# Autodesk Inventor assembly: ASY MSC 100 cone
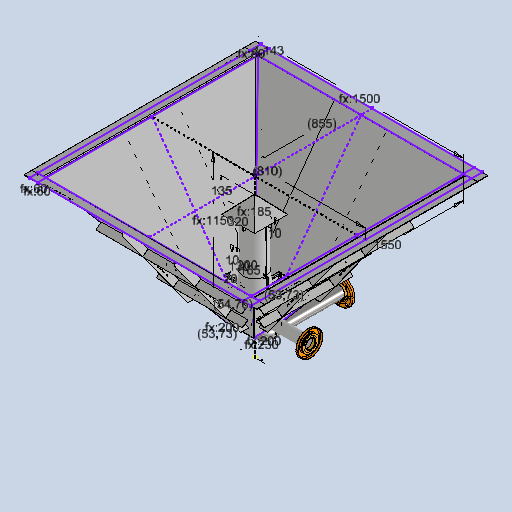
[picture p0: Inventor's stored thumbnail of the model, 512x512]
Saved by Autodesk Inventor 2025 (Build 290162010, 162A)
## iProperties
Created: 2024-05-19
Part Number: ASY MSC 100 cone
Document SubType Name: Assembly
Designer: admin
Mass: 170206 g
Surface Area: 120081 cm^2
Volume: 21304.1 cm^3
Density: 7.98935 g/cm^3
Stock Number: ASY МОО 100 конус
Author: admin
## Documents named in this file (17)
- C:\Users\pokla\Documents\Inventor\Отстойник осветлитель\Manturovo_Se-clar-Gleb\ASY MSC 100 cone.iam
- C:\Users\pokla\Documents\Inventor\Отстойник осветлитель\Manturovo_Se-clar-Gleb\MSC 114 cone IN right board.ipt
- C:\Users\pokla\Documents\Inventor\Отстойник осветлитель\Manturovo_Se-clar-Gleb\MSC 111 cone IN bottom.ipt
- C:\Users\pokla\Documents\Inventor\Отстойник осветлитель\Manturovo_Se-clar-Gleb\MSC 113 cone IN left board.ipt
- C:\Users\pokla\Documents\Inventor\Отстойник осветлитель\Manturovo_Se-clar-Gleb\MSC 112 cone IN back.ipt
- C:\Users\pokla\Documents\Inventor\Отстойник осветлитель\Manturovo_Se-clar-Gleb\MSC DIM 001 cone sketch.ipt
- C:\Users\pokla\Documents\Inventor\Отстойник осветлитель\Manturovo_Se-clar-Gleb\MSC 115 cone IN bow.ipt
- C:\Users\pokla\Documents\Inventor\Отстойник осветлитель\Manturovo_Se-clar-Gleb\MSC 110 stringer cone.ipt
- C:\Users\pokla\Documents\Inventor\Отстойник осветлитель\Manturovo_Se-clar-Gleb\MSC 106 rib cone.ipt
- C:\Users\pokla\Documents\Inventor\Отстойник осветлитель\Manturovo_Se-clar-Gleb\MSC 107 rib cone.ipt
- C:\Users\pokla\Documents\Inventor\Отстойник осветлитель\Manturovo_Se-clar-Gleb\MSC 108 rib cone.ipt
- C:\Users\pokla\Documents\Inventor\Отстойник осветлитель\Manturovo_Se-clar-Gleb\MSC 109 rib cone.ipt
- C:\Users\pokla\Documents\Inventor\Отстойник осветлитель\Manturovo_Se-clar-Gleb\ASY MSC 100.2 Cone tube.iam
- C:\Users\pokla\Documents\Inventor\Отстойник осветлитель\Manturovo_Se-clar-Gleb\ASY MSC 100.1 roсket.iam
- C:\Users\pokla\Documents\Inventor\Отстойник осветлитель\Manturovo_Se-clar-Gleb\MSC 116 rocket tube 8.ipt
- C:\Users\pokla\Documents\Inventor\Отстойник осветлитель\Manturovo_Se-clar-Gleb\Stamp flange DIN2642-065.ipt
- C:\Users\pokla\Documents\Inventor\Отстойник осветлитель\Manturovo_Se-clar-Gleb\3d party\Stamp flange DIN2642\Stamd flange lapped collar DIN2642.ipt
## Components (26 placed, 15 different names)
1. MSC DIM 001 cone sketch.ipt:1 — Flush:8, Flush:9, Mate:1
2. MSC 112 cone IN back.ipt:1 — Flush:6, Flush:10, Mate:2, Mate:49, Mate:70, Mate:72
3. MSC 111 cone IN bottom.ipt:1 — Flush:4, Flush:5, Flush:11, Rigid:1
4. MSC 114 cone IN right board.ipt:1 — Flush:13, Flush:15, Mate:63, Mate:66, Mate:67, Mate:68, Mate:69, Flush:18
5. MSC 113 cone IN left board.ipt:1 — Mate:4, Flush:14, Mate:5
6. MSC 115 cone IN bow.ipt:1 — Mate:3, Mate:6, Flush:16, Flush:17
7. ASY MSC 100.1 roсket.iam:1 [sub-assembly] — Rigid:2
8. ASY MSC 100.2 Cone tube.iam:1 [sub-assembly] — Rigid:1, Rigid:2
9. MSC 116 rocket tube 8.ipt:1 — Rigid:3
10. Stamp flange DIN2642-065.ipt:1 — Rigid:3
11. MSC 110 stringer cone.ipt:1 — Rigid:7
12. MSC 107 rib cone.ipt:1 — Rigid:9
13. MSC 110 stringer cone.ipt:2 — Mate:49, Rigid:8, Rigid:9, Mate:72
14. MSC 110 stringer cone.ipt:3 — Rigid:5
15. MSC 108 rib cone.ipt:1 — Mate:66, Rigid:4, Rigid:5, Mate:67, Mate:68
16. MSC 110 stringer cone.ipt:4 — Rigid:4, Rigid:6, Mate:69
17. MSC 109 rib cone.ipt:1 — Mate:63, Rigid:6
18. MSC 106 rib cone.ipt:1 — Rigid:7, Rigid:8, Mate:70, Mate:71
19. MSC 110 stringer cone.ipt:5
20. MSC 107 rib cone.ipt:2
21. MSC 110 stringer cone.ipt:6
22. MSC 110 stringer cone.ipt:7
23. MSC 108 rib cone.ipt:2
24. MSC 110 stringer cone.ipt:8
25. MSC 109 rib cone.ipt:2
26. MSC 106 rib cone.ipt:2
## Component patterns: (2 elements, first: MSC 110 stringer cone.ipt:1 + MSC 107 rib cone.ipt:1 + MSC 110 stringer cone.ipt:2 + MSC 110 stringer cone.ipt:3 + MSC 108 rib cone.ipt:1 + MSC 110 stringer cone.ipt:4 + MSC 109 rib cone.ipt:1 + MSC 106 rib cone.ipt:1)
## Relationships (38: Mate 15, Flush 13, WeldJoint 9, CylindricalJoint 1)
- Flush:4: MSC 111 cone IN bottom.ipt:1
- Flush:5: MSC 111 cone IN bottom.ipt:1
- Flush:6: MSC 112 cone IN back.ipt:1
- Flush:8: MSC DIM 001 cone sketch.ipt:1
- Flush:9: MSC DIM 001 cone sketch.ipt:1
- Mate:1: MSC DIM 001 cone sketch.ipt:1
- Flush:10: MSC 112 cone IN back.ipt:1
- Mate:2: MSC 112 cone IN back.ipt:1
- Flush:11 (-230 mm): MSC 111 cone IN bottom.ipt:1
- Mate:3: MSC 115 cone IN bow.ipt:1
- Flush:13: MSC 114 cone IN right board.ipt:1
- Mate:4: MSC 113 cone IN left board.ipt:1
- Flush:14: MSC 113 cone IN left board.ipt:1
- Mate:5: MSC 113 cone IN left board.ipt:1
- Flush:15: MSC 114 cone IN right board.ipt:1
- Mate:6: MSC 115 cone IN bow.ipt:1
- Flush:16: MSC 115 cone IN bow.ipt:1
- Flush:17: MSC 115 cone IN bow.ipt:1
- Mate:49: MSC 112 cone IN back.ipt:1 ↔ MSC 110 stringer cone.ipt:2
- Mate:63: MSC 114 cone IN right board.ipt:1 ↔ MSC 109 rib cone.ipt:1
- Mate:66: MSC 114 cone IN right board.ipt:1 ↔ MSC 108 rib cone.ipt:1
- Rigid:1 [WeldJoint]: MSC 111 cone IN bottom.ipt:1 ↔ ASY MSC 100.2 Cone tube.iam:1
- Rigid:2 [WeldJoint] (50 mm): ASY MSC 100.1 roсket.iam:1 ↔ ASY MSC 100.2 Cone tube.iam:1
- [CylindricalJoint]: MSC 113 cone IN left board.ipt:1 ↔ MSC 116 rocket tube 8.ipt:1
- Rigid:3 [WeldJoint]: MSC 116 rocket tube 8.ipt:1 ↔ Stamp flange DIN2642-065.ipt:1
- Rigid:4 [WeldJoint] (2 mm): MSC 108 rib cone.ipt:1 ↔ MSC 110 stringer cone.ipt:4
- Rigid:5 [WeldJoint] (2 mm): MSC 110 stringer cone.ipt:3 ↔ MSC 108 rib cone.ipt:1
- Rigid:6 [WeldJoint] (2 mm): MSC 110 stringer cone.ipt:4 ↔ MSC 109 rib cone.ipt:1
- Mate:67: MSC 114 cone IN right board.ipt:1 ↔ MSC 108 rib cone.ipt:1
- Mate:68: MSC 114 cone IN right board.ipt:1 ↔ MSC 108 rib cone.ipt:1
- Mate:69 (5 mm): MSC 114 cone IN right board.ipt:1 ↔ MSC 110 stringer cone.ipt:4
- Rigid:7 [WeldJoint] (3 mm): MSC 110 stringer cone.ipt:1 ↔ MSC 106 rib cone.ipt:1
- Rigid:8 [WeldJoint] (2 mm): MSC 110 stringer cone.ipt:2 ↔ MSC 106 rib cone.ipt:1
- Rigid:9 [WeldJoint] (2 mm): MSC 107 rib cone.ipt:1 ↔ MSC 110 stringer cone.ipt:2
- Mate:70: MSC 112 cone IN back.ipt:1 ↔ MSC 106 rib cone.ipt:1
- Flush:18: MSC 114 cone IN right board.ipt:1
- Mate:71: MSC 106 rib cone.ipt:1
- Mate:72 (5 mm): MSC 112 cone IN back.ipt:1 ↔ MSC 110 stringer cone.ipt:2
